# Autodesk Inventor assembly: 机架one
Saved by Autodesk Inventor 2013 (Build 170138000, 138)
## iProperties
Created: 2012-04-28
Part Number: 机架one
Document SubType Name: Assembly
Designer: Zhensheng
Author: Zhensheng
## Documents named in this file (3)
- E:\inventor\插床概念草图\机架one.iam
- E:\inventor\插床概念草图\机架one_Layout.ipt
- E:\inventor\插床概念草图\机架1.ipt
## Components (3 placed, 2 different names)
1. 机架one_Layout:1
2. 机架1:1
3. 机架1:2
## Relationships (2: Composite 2)
- [Composite]: 机架one_Layout:1 ↔ 机架1:1
- [Composite]: 机架one_Layout:1 ↔ 机架1:2
